# Autodesk Inventor assembly: 페그보드 조립
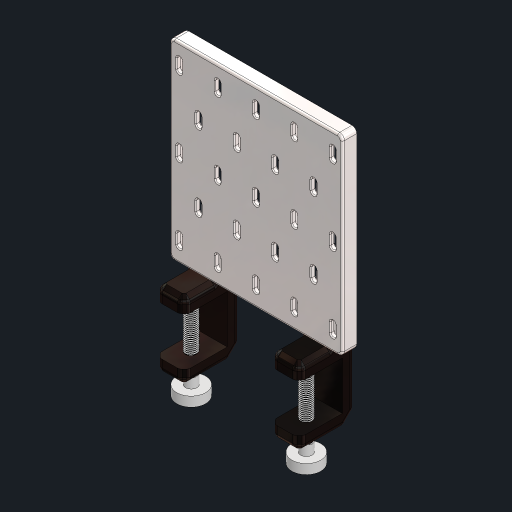
[picture p0: Inventor's stored thumbnail of the model, 512x512]
Saved by Autodesk Inventor 2024 (Build 280153000, 153)
## iProperties
Created: 2024-02-06
Part Number: 페그보드 조립
Document SubType Name: Assembly
Designer: KBU
Author: KBU
## Documents named in this file (6)
- D:\github\Modeling\IKEA 페그보드 시제품\페그보드 조립.iam
- D:\github\Modeling\IKEA 페그보드 시제품\SKÅDIS Pegboard Clamp.ipt
- D:\github\Modeling\IKEA 페그보드 시제품\SKÅDIS Pegboard.ipt
- D:\github\Modeling\IKEA 페그보드 시제품\SKÅDIS Pegboard Clamp1.ipt
- D:\github\Modeling\IKEA 페그보드 시제품\SKÅDIS Pegboard Clamp2.ipt
- D:\github\Modeling\IKEA 페그보드 시제품\SKÅDIS Pegboard Clamp Screw.ipt
## Components (8 placed, 5 different names)
1. SKÅDIS Pegboard Clamp:1 — 메이트:1, 플러쉬:1
2. SKÅDIS Pegboard:1 — 메이트:1, 플러쉬:1, 메이트:2, 플러쉬:2, 메이트:7, 플러쉬:5
3. SKÅDIS Pegboard Clamp1:1 — 메이트:2, 플러쉬:2, 메이트:3, 플러쉬:3, 메이트:4
4. SKÅDIS Pegboard Clamp2:1 — 메이트:3, 플러쉬:3, 메이트:4, 원통형:2
5. SKÅDIS Pegboard Clamp1:2 — 메이트:7, 플러쉬:5
6. SKÅDIS Pegboard Clamp2:2 — 원통형:1
7. SKÅDIS Pegboard Clamp Screw:1 — 원통형:1
8. SKÅDIS Pegboard Clamp Screw:2 — 원통형:2
## Relationships (14: Mate 7, Flush 5, CylindricalJoint 2)
- 메이트:1 [Mate]: SKÅDIS Pegboard Clamp:1 ↔ SKÅDIS Pegboard:1
- 플러쉬:1 [Flush]: SKÅDIS Pegboard Clamp:1 ↔ SKÅDIS Pegboard:1
- 메이트:2 [Mate]: SKÅDIS Pegboard:1 ↔ SKÅDIS Pegboard Clamp1:1
- 플러쉬:2 [Flush]: SKÅDIS Pegboard:1 ↔ SKÅDIS Pegboard Clamp1:1
- 메이트:3 [Mate] (0.05 mm): SKÅDIS Pegboard Clamp1:1 ↔ SKÅDIS Pegboard Clamp2:1
- 플러쉬:3 [Flush]: SKÅDIS Pegboard Clamp1:1 ↔ SKÅDIS Pegboard Clamp2:1
- 메이트:4 [Mate] (0.1 mm): SKÅDIS Pegboard Clamp1:1 ↔ SKÅDIS Pegboard Clamp2:1
- [Mate] (0.05 mm): SKÅDIS Pegboard Clamp1:2 ↔ SKÅDIS Pegboard Clamp2:2
- [Flush]: SKÅDIS Pegboard Clamp1:2 ↔ SKÅDIS Pegboard Clamp2:2
- [Mate] (0.1 mm): SKÅDIS Pegboard Clamp1:2 ↔ SKÅDIS Pegboard Clamp2:2
- 메이트:7 [Mate]: SKÅDIS Pegboard:1 ↔ SKÅDIS Pegboard Clamp1:2
- 플러쉬:5 [Flush]: SKÅDIS Pegboard:1 ↔ SKÅDIS Pegboard Clamp1:2
- 원통형:1 [CylindricalJoint]: SKÅDIS Pegboard Clamp2:2 ↔ SKÅDIS Pegboard Clamp Screw:1
- 원통형:2 [CylindricalJoint]: SKÅDIS Pegboard Clamp2:1 ↔ SKÅDIS Pegboard Clamp Screw:2
## Named parameters: d27_d23 = 0.05 mm, d28_d24 = 0 mm, d29_d25 = 0.1 mm
